# Autodesk Inventor assembly: gimbal_assembly_3
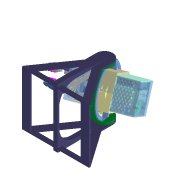
[picture p0: Inventor's stored thumbnail of the model, 180x180]
Saved by Autodesk Inventor 2022 (Build 260153000, 153)
## iProperties
Created: 2022-03-15
Part Number: gimbal_assembly_3
Document SubType Name: Assembly
Designer: kylem
Author: kylem
## Documents named in this file (7)
- C:\Users\kylem\OneDrive\Documents\GitHub\IMML_Contactile_Gripper_Hardware\gimbal_assembly_3.iam
- C:\Users\kylem\OneDrive\Documents\GitHub\IMML_Contactile_Gripper_Hardware\Gripper_Design_NonCompliant_No_UR5.iam
- C:\Users\kylem\OneDrive\Documents\GitHub\IMML_Contactile_Gripper_Hardware\test_stand\gripper_mount_female.ipt
- C:\Users\kylem\OneDrive\Documents\GitHub\IMML_Contactile_Gripper_Hardware\test_stand\gripper_mount_male.ipt
- C:\Users\kylem\OneDrive\Documents\GitHub\IMML_Contactile_Gripper_Hardware\test_stand\gripper_mount_ring.ipt
- C:\Users\kylem\OneDrive\Documents\GitHub\IMML_Contactile_Gripper_Hardware\bottom_gimbal_ring_3.ipt
- C:\Users\kylem\OneDrive\Documents\GitHub\IMML_Contactile_Gripper_Hardware\test_stand\gimbal_ring_second_2.ipt
## Components (6 placed, 6 different names)
1. Gripper_Design_NonCompliant_No_UR5:1 [sub-assembly] — Mate:12, Mate:13, Mate:14, Mate:17
2. gripper_mount_female:1 — Mate:12, Mate:13, Mate:14, Mate:15, Mate:16
3. gripper_mount_male:1 — Mate:15, Mate:16, Mate:17, Mate:22, Mate:24, Mate:33, Mate:37
4. gripper_mount_ring:1 — Mate:22, Mate:24, Mate:32, Mate:37
5. bottom_gimbal_ring_3:1 — Mate:29, Mate:30, Mate:34, Mate:35, Mate:36
6. gimbal_ring_second_2:1 — Mate:32, Mate:33, Mate:34, Mate:36
## Relationships (16: Mate 16)
- Mate:12: Gripper_Design_NonCompliant_No_UR5:1 ↔ gripper_mount_female:1
- Mate:13: Gripper_Design_NonCompliant_No_UR5:1 ↔ gripper_mount_female:1
- Mate:14: Gripper_Design_NonCompliant_No_UR5:1 ↔ gripper_mount_female:1
- Mate:15: gripper_mount_female:1 ↔ gripper_mount_male:1
- Mate:16: gripper_mount_female:1 ↔ gripper_mount_male:1
- Mate:17: Gripper_Design_NonCompliant_No_UR5:1 ↔ gripper_mount_male:1
- Mate:22: gripper_mount_male:1 ↔ gripper_mount_ring:1
- Mate:24: gripper_mount_male:1 ↔ gripper_mount_ring:1
- Mate:29: bottom_gimbal_ring_3:1
- Mate:30: bottom_gimbal_ring_3:1
- Mate:32: gripper_mount_ring:1 ↔ gimbal_ring_second_2:1
- Mate:33 (0.25 mm): gripper_mount_male:1 ↔ gimbal_ring_second_2:1
- Mate:34: bottom_gimbal_ring_3:1 ↔ gimbal_ring_second_2:1
- Mate:35: bottom_gimbal_ring_3:1
- Mate:36: bottom_gimbal_ring_3:1 ↔ gimbal_ring_second_2:1
- Mate:37: gripper_mount_male:1 ↔ gripper_mount_ring:1
